# Autodesk Inventor assembly: Intakewchain
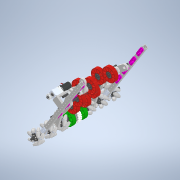
[picture p0: Inventor's stored thumbnail of the model, 180x180]
Saved by Autodesk Inventor 2020 (Build 240168000, 168)
## iProperties
Created: 2020-01-19
Part Number: Intakewchain
Document SubType Name: Assembly
Designer: srini
Author: srini
## Documents named in this file (17)
- C:\Users\srini\Documents\FRC\2020\IntakeShooter\Intakewchain.iam
- C:\Users\srini\Documents\FRC\2020\IntakeShooter\ChainLinkWBearings.iam
- C:\Users\srini\Documents\FRC\2020\IntakeShooter\ChainLinkEndWBearings.iam
- C:\Users\srini\Documents\FRC\2020\IntakeShooter\1_4_Acetal_Spacer_-_1_2_Hex_217-3259.ipt
- C:\Users\srini\Documents\FRC\2020\IntakeShooter\am-3999 17T 25 Chain Double Sprocket For WCD.ipt
- C:\Users\srini\Documents\FRC\2020\ThunderHex_27in.ipt
- C:\Users\srini\Documents\FRC\2020\am-2256 4 in HiGrip Wheel_HexBore.iam
- C:\Users\srini\Documents\FRC\2020\am-3480 4IN 500Hex Compliant Wheel REV2.iam
- C:\Users\srini\Documents\FRC\2020\MecWheels\4_Mecanum_Wheel_Left_217-3644.iam
- C:\Users\srini\Documents\FRC\2020\MecWheels\4_Mecanum_Wheel_Right_217-3645.iam
- C:\Users\srini\Documents\FRC\2020\am-3480 4IN 500Hex Compliant Wheel REV2_Black.iam
- C:\Users\srini\Documents\FRC\2020\IntakeShooter\ChainlinkVP.iam
- C:\Users\srini\Documents\FRC\2020\IntakeShooter\VersaPlanetary_v2_Two_Stage_100_1_with_BAG.iam
- C:\Users\srini\Documents\FRC\2020\IntakeShooter\IntakeExtensionBar.iam
- C:\Users\srini\Documents\FRC\2020\ThunderHex_16in.ipt
- C:\Users\srini\Documents\FRC\2020\ThunderHex_6in.ipt
- C:\Users\srini\Documents\FRC\2020\IntakeShooter\IntakeExtensionBar_MIR1.iam
## Components (54 placed, 16 different names)
1. ChainLinkWBearings:2 [sub-assembly] — Insert:4, Insert:5, Insert:13, Insert:29
2. 1_4_Acetal_Spacer_-_1_2_Hex_217-3259:1 — Insert:4, Insert:7
3. 1_4_Acetal_Spacer_-_1_2_Hex_217-3259:2 — Insert:5, Insert:8
4. 1_4_Acetal_Spacer_-_1_2_Hex_217-3259:3 — Insert:9, Insert:42
5. am-3999 17T 25 Chain Double Sprocket For WCD:1 — Insert:7, Insert:10, Insert:16
6. am-3999 17T 25 Chain Double Sprocket For WCD:2 — Insert:8, Flush:1, Insert:50
7. am-3999 17T 25 Chain Double Sprocket For WCD:3 — Insert:9, Insert:51
8. ThunderHex_27in:1 — Insert:10
9. am-2256 4 in HiGrip Wheel_HexBore:1 [sub-assembly] — Insert:12, Insert:15
10. am-3480 4IN 500Hex Compliant Wheel REV2:1 [sub-assembly] — Insert:12, Insert:14
11. am-3480 4IN 500Hex Compliant Wheel REV2:2 [sub-assembly] — Insert:15, Insert:17
12. 4_Mecanum_Wheel_Left_217-3644:1 [sub-assembly] — Insert:13, Insert:14
13. 4_Mecanum_Wheel_Left_217-3644:2 [sub-assembly] — Insert:16, Insert:33
14. 4_Mecanum_Wheel_Left_217-3644:3 [sub-assembly] — Insert:40
15. 4_Mecanum_Wheel_Right_217-3645:1 [sub-assembly] — Insert:17, Insert:18
16. 4_Mecanum_Wheel_Right_217-3645:2 [sub-assembly] — Insert:73
17. 4_Mecanum_Wheel_Right_217-3645:3 [sub-assembly] — Insert:21, Insert:72
18. ChainLinkWBearings:3 [sub-assembly] — Insert:18, Insert:19, Insert:21
19. ChainLinkWBearings:4 [sub-assembly] — Insert:19, Insert:27, Insert:28, Mate:5, Mate:6, Insert:43
20. am-3480 4IN 500Hex Compliant Wheel REV2_Black:1 [sub-assembly] — Insert:36
21. am-3480 4IN 500Hex Compliant Wheel REV2_Black:2 [sub-assembly] — Insert:35
22. am-3480 4IN 500Hex Compliant Wheel REV2_Black:3 [sub-assembly] — Insert:27
23. am-3480 4IN 500Hex Compliant Wheel REV2_Black:4 [sub-assembly] — Insert:28
24. ChainlinkVP:1 [sub-assembly] — Insert:29, Insert:31, Insert:32, Insert:35, Insert:36, Mate:5, Mate:6, Insert:41
25. VersaPlanetary_v2_Two_Stage_100_1_with_BAG:1 [sub-assembly] — Insert:31, Insert:32, Mate:4
26. am-3999 17T 25 Chain Double Sprocket For WCD:4 — Mate:4, Flush:1
27. IntakeExtensionBar:2 [sub-assembly] — Insert:33, Insert:40, Flush:2
28. ChainLinkWBearings:5 [sub-assembly] — Insert:41, Insert:42, Insert:48, Insert:54
29. ChainLinkWBearings:6 [sub-assembly] — Insert:43, Insert:55, Insert:68, Insert:69
30. am-3480 4IN 500Hex Compliant Wheel REV2_Black:5 [sub-assembly] — Insert:52, Insert:58, Mate:8
31. am-3480 4IN 500Hex Compliant Wheel REV2_Black:6 [sub-assembly] — Insert:53, Insert:59, Mate:8
32. am-3999 17T 25 Chain Double Sprocket For WCD:5 — Insert:49
33. 1_4_Acetal_Spacer_-_1_2_Hex_217-3259:4 — Insert:48, Insert:49
34. ThunderHex_16in:1 — Insert:50
35. ThunderHex_16in:2 — Insert:51
36. ThunderHex_6in:1 — Insert:53
37. ThunderHex_6in:2 — Insert:52
38. ChainLinkWBearings:7 [sub-assembly] — Insert:55, Insert:59, Insert:61, Insert:64
39. ChainLinkWBearings:8 [sub-assembly] — Insert:54, Insert:58, Insert:60, Insert:63
40. am-3480 4IN 500Hex Compliant Wheel REV2_Black:7 [sub-assembly] — Insert:60, Mate:7
41. ThunderHex_6in:3
42. am-3480 4IN 500Hex Compliant Wheel REV2_Black:8 [sub-assembly] — Insert:61, Mate:7
43. ThunderHex_6in:4
44. ChainLinkEndWBearings:1 [sub-assembly] — Insert:63, Insert:65
45. ChainLinkEndWBearings:2 [sub-assembly] — Insert:64, Insert:71
46. am-3999 17T 25 Chain Double Sprocket For WCD:6
47. 1_4_Acetal_Spacer_-_1_2_Hex_217-3259:5 — Insert:65
48. am-3999 17T 25 Chain Double Sprocket For WCD:7
49. 1_4_Acetal_Spacer_-_1_2_Hex_217-3259:6 — Insert:69
50. am-3999 17T 25 Chain Double Sprocket For WCD:8
51. 1_4_Acetal_Spacer_-_1_2_Hex_217-3259:7 — Insert:68
52. am-3999 17T 25 Chain Double Sprocket For WCD:9
53. 1_4_Acetal_Spacer_-_1_2_Hex_217-3259:8 — Insert:71
54. IntakeExtensionBar_MIR1:1 [sub-assembly] — Insert:72, Insert:73, Flush:2
## Relationships (60: Insert 53, Mate 5, Flush 2)
- Insert:4: ChainLinkWBearings:2 ↔ 1_4_Acetal_Spacer_-_1_2_Hex_217-3259:1
- Insert:5: ChainLinkWBearings:2 ↔ 1_4_Acetal_Spacer_-_1_2_Hex_217-3259:2
- Insert:7: 1_4_Acetal_Spacer_-_1_2_Hex_217-3259:1 ↔ am-3999 17T 25 Chain Double Sprocket For WCD:1
- Insert:8: 1_4_Acetal_Spacer_-_1_2_Hex_217-3259:2 ↔ am-3999 17T 25 Chain Double Sprocket For WCD:2
- Insert:9: 1_4_Acetal_Spacer_-_1_2_Hex_217-3259:3 ↔ am-3999 17T 25 Chain Double Sprocket For WCD:3
- Insert:10 (165.1 mm): am-3999 17T 25 Chain Double Sprocket For WCD:1 ↔ ThunderHex_27in:1
- Insert:12 (12.7 mm): am-2256 4 in HiGrip Wheel_HexBore:1 ↔ am-3480 4IN 500Hex Compliant Wheel REV2:1
- Insert:13 (3.175 mm): ChainLinkWBearings:2 ↔ 4_Mecanum_Wheel_Left_217-3644:1
- Insert:14 (12.7 mm): am-3480 4IN 500Hex Compliant Wheel REV2:1 ↔ 4_Mecanum_Wheel_Left_217-3644:1
- Insert:15 (12.7 mm): am-2256 4 in HiGrip Wheel_HexBore:1 ↔ am-3480 4IN 500Hex Compliant Wheel REV2:2
- Insert:16: am-3999 17T 25 Chain Double Sprocket For WCD:1 ↔ 4_Mecanum_Wheel_Left_217-3644:2
- Insert:17 (12.7 mm): am-3480 4IN 500Hex Compliant Wheel REV2:2 ↔ 4_Mecanum_Wheel_Right_217-3645:1
- Insert:18 (3.175 mm): 4_Mecanum_Wheel_Right_217-3645:1 ↔ ChainLinkWBearings:3
- Insert:19: ChainLinkWBearings:3 ↔ ChainLinkWBearings:4
- Insert:21 (19.05 mm): 4_Mecanum_Wheel_Right_217-3645:3 ↔ ChainLinkWBearings:3
- Insert:27 (57.15 mm): ChainLinkWBearings:4 ↔ am-3480 4IN 500Hex Compliant Wheel REV2_Black:3
- Insert:28 (44.45 mm): ChainLinkWBearings:4 ↔ am-3480 4IN 500Hex Compliant Wheel REV2_Black:4
- Insert:29: ChainLinkWBearings:2 ↔ ChainlinkVP:1
- Insert:31: ChainlinkVP:1 ↔ VersaPlanetary_v2_Two_Stage_100_1_with_BAG:1
- Insert:32: ChainlinkVP:1 ↔ VersaPlanetary_v2_Two_Stage_100_1_with_BAG:1
- Mate:4: VersaPlanetary_v2_Two_Stage_100_1_with_BAG:1 ↔ am-3999 17T 25 Chain Double Sprocket For WCD:4
- Flush:1: am-3999 17T 25 Chain Double Sprocket For WCD:2 ↔ am-3999 17T 25 Chain Double Sprocket For WCD:4
- Insert:33 (3.175 mm): 4_Mecanum_Wheel_Left_217-3644:2 ↔ IntakeExtensionBar:2
- Insert:35 (57.15 mm): am-3480 4IN 500Hex Compliant Wheel REV2_Black:2 ↔ ChainlinkVP:1
- Insert:36 (44.45 mm): am-3480 4IN 500Hex Compliant Wheel REV2_Black:1 ↔ ChainlinkVP:1
- Insert:40 (3.175 mm): 4_Mecanum_Wheel_Left_217-3644:3 ↔ IntakeExtensionBar:2
- Mate:5: ChainLinkWBearings:4 ↔ ChainlinkVP:1
- Mate:6: ChainLinkWBearings:4 ↔ ChainlinkVP:1
- Insert:41: ChainlinkVP:1 ↔ ChainLinkWBearings:5
- Insert:42: 1_4_Acetal_Spacer_-_1_2_Hex_217-3259:3 ↔ ChainLinkWBearings:5
- Insert:43: ChainLinkWBearings:4 ↔ ChainLinkWBearings:6
- Insert:48: ChainLinkWBearings:5 ↔ 1_4_Acetal_Spacer_-_1_2_Hex_217-3259:4
- Insert:49: am-3999 17T 25 Chain Double Sprocket For WCD:5 ↔ 1_4_Acetal_Spacer_-_1_2_Hex_217-3259:4
- Insert:50 (-38.1 mm): am-3999 17T 25 Chain Double Sprocket For WCD:2 ↔ ThunderHex_16in:1
- Insert:51 (-38.1 mm): am-3999 17T 25 Chain Double Sprocket For WCD:3 ↔ ThunderHex_16in:2
- Insert:52 (-6.35 mm): am-3480 4IN 500Hex Compliant Wheel REV2_Black:5 ↔ ThunderHex_6in:2
- Insert:53 (-6.35 mm): am-3480 4IN 500Hex Compliant Wheel REV2_Black:6 ↔ ThunderHex_6in:1
- Insert:54: ChainLinkWBearings:5 ↔ ChainLinkWBearings:8
- Insert:55: ChainLinkWBearings:6 ↔ ChainLinkWBearings:7
- [Insert] (-6.35 mm): am-3480 4IN 500Hex Compliant Wheel REV2_Black:7 ↔ ThunderHex_6in:3
- [Insert] (-6.35 mm): am-3480 4IN 500Hex Compliant Wheel REV2_Black:8 ↔ ThunderHex_6in:4
- Insert:58 (25.4 mm): am-3480 4IN 500Hex Compliant Wheel REV2_Black:5 ↔ ChainLinkWBearings:8
- Insert:59 (25.4 mm): am-3480 4IN 500Hex Compliant Wheel REV2_Black:6 ↔ ChainLinkWBearings:7
- Insert:60 (25.4 mm): ChainLinkWBearings:8 ↔ am-3480 4IN 500Hex Compliant Wheel REV2_Black:7
- Insert:61 (25.4 mm): ChainLinkWBearings:7 ↔ am-3480 4IN 500Hex Compliant Wheel REV2_Black:8
- [Insert]: am-3999 17T 25 Chain Double Sprocket For WCD:6 ↔ 1_4_Acetal_Spacer_-_1_2_Hex_217-3259:5
- Insert:63: ChainLinkWBearings:8 ↔ ChainLinkEndWBearings:1
- Insert:64: ChainLinkWBearings:7 ↔ ChainLinkEndWBearings:2
- Insert:65: ChainLinkEndWBearings:1 ↔ 1_4_Acetal_Spacer_-_1_2_Hex_217-3259:5
- [Insert]: am-3999 17T 25 Chain Double Sprocket For WCD:7 ↔ 1_4_Acetal_Spacer_-_1_2_Hex_217-3259:6
- [Insert]: am-3999 17T 25 Chain Double Sprocket For WCD:8 ↔ 1_4_Acetal_Spacer_-_1_2_Hex_217-3259:7
- Insert:68: ChainLinkWBearings:6 ↔ 1_4_Acetal_Spacer_-_1_2_Hex_217-3259:7
- Insert:69: ChainLinkWBearings:6 ↔ 1_4_Acetal_Spacer_-_1_2_Hex_217-3259:6
- [Insert]: am-3999 17T 25 Chain Double Sprocket For WCD:9 ↔ 1_4_Acetal_Spacer_-_1_2_Hex_217-3259:8
- Insert:71: ChainLinkEndWBearings:2 ↔ 1_4_Acetal_Spacer_-_1_2_Hex_217-3259:8
- Insert:72 (3.175 mm): 4_Mecanum_Wheel_Right_217-3645:3 ↔ IntakeExtensionBar_MIR1:1
- Insert:73 (3.175 mm): 4_Mecanum_Wheel_Right_217-3645:2 ↔ IntakeExtensionBar_MIR1:1
- Flush:2: IntakeExtensionBar:2 ↔ IntakeExtensionBar_MIR1:1
- Mate:7: am-3480 4IN 500Hex Compliant Wheel REV2_Black:7 ↔ am-3480 4IN 500Hex Compliant Wheel REV2_Black:8
- Mate:8: am-3480 4IN 500Hex Compliant Wheel REV2_Black:5 ↔ am-3480 4IN 500Hex Compliant Wheel REV2_Black:6
## Named parameters: d67_d63 = -6.35 mm, d68_d64 = -6.35 mm, d73_d59 = 0 mm, d77_d59 = 0 mm, d78_d59 = 0 mm, d81_d59 = 0 mm
